# Autodesk Inventor assembly: ensambaje
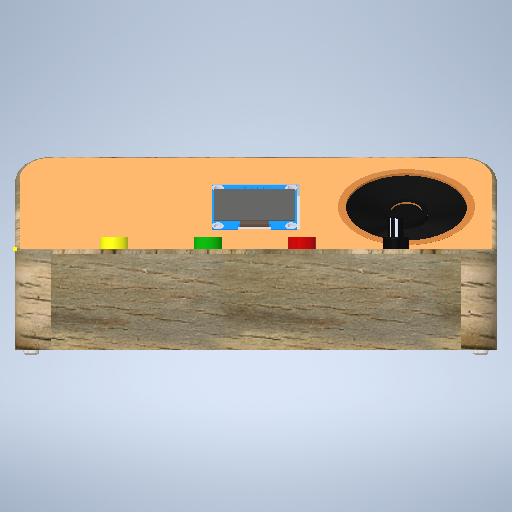
[picture p0: Inventor's stored thumbnail of the model, 512x512]
Saved by Autodesk Inventor 2025.3 (Build 293356000, 356)
## iProperties
Created: 2025-12-16
Part Number: ensambaje
Document SubType Name: Assembly
Designer: ar287
Author: ar287
## Documents named in this file (12)
- C:\Users\ar287\OneDrive - Escuela Superior Politécnica del Litoral\EMBEBIDOS\tarea4\ensambaje.iam
- C:\Users\ar287\OneDrive - Escuela Superior Politécnica del Litoral\EMBEBIDOS\tarea4\base.ipt
- C:\Users\ar287\Downloads\oled-1-3-128x64-1.snapshot.10\step\oled\oled\oledoled.ipt
- C:\Users\ar287\Downloads\bocina_57mm-1.snapshot.1\Bocina_57mm\Bocina_57mm\bocinaBocina_57mm.ipt
- C:\Users\ar287\OneDrive - Escuela Superior Politécnica del Litoral\EMBEBIDOS\tarea4\boton amarillo.ipt
- C:\Users\ar287\OneDrive - Escuela Superior Politécnica del Litoral\EMBEBIDOS\tarea4\boton rojo.ipt
- C:\Users\ar287\OneDrive - Escuela Superior Politécnica del Litoral\EMBEBIDOS\tarea4\boton verde.ipt
- C:\Users\ar287\OneDrive - Escuela Superior Politécnica del Litoral\EMBEBIDOS\tarea4\estuche de pot.ipt
- C:\Users\ar287\OneDrive - Escuela Superior Politécnica del Litoral\EMBEBIDOS\tarea4\pot.ipt
- C:\Users\ar287\Downloads\esp32-c6-wroom-1-1.snapshot.2\ESP32C6\ESP32C6\espESP32C6.iam
- C:\Users\ar287\Downloads\dfplayer-mini-3.snapshot.1\DFPlayer Mini Assem v1\DFPlayer Mini Assem v1\dfDFPlayer Mini Assem v1.iam
- C:\Users\ar287\OneDrive\Documentos\Inventor\Content Center Files\R2025\es-ES\DIN 7985 (Z)\DIN 7985 (Z) - M2,5x3-Z.ipt
## Components (21 placed, 11 different names)
1. base:1 — Coincidencia:1, Coincidencia:2, Coincidencia:3, Insertar:1, Coincidencia:4, Coincidencia:5, Nivelación:1, Insertar:2, Nivelación:2, Insertar:3, Nivelación:3, Insertar:4, Coincidencia:7, Insertar:6, Coincidencia:8, Coincidencia:9, Coincidencia:10, Coincidencia:11, Coincidencia:12, Coincidencia:13, Insertar:7, Insertar:8, Insertar:9, Insertar:10, Insertar:11, Coincidencia:14, Coincidencia:15, Coincidencia:16, Coincidencia:17, Coincidencia:18, Coincidencia:19, Coincidencia:20, Coincidencia:21, Coincidencia:22, Coincidencia:23, Coincidencia:24, Coincidencia:25
2. oledoled:1 — Coincidencia:1, Coincidencia:2, Coincidencia:3, Coincidencia:5
3. bocinaBocina_57mm:1 — Insertar:1, Coincidencia:4
4. boton amarillo:1 — Nivelación:1, Insertar:2
5. boton rojo:1 — Nivelación:3, Insertar:4
6. boton verde:1 — Nivelación:2, Insertar:3
7. estuche de pot:1 — Coincidencia:6, Insertar:5, Coincidencia:7, Insertar:6
8. pot:1 — Coincidencia:6, Insertar:5
9. espESP32C6:1 [sub-assembly] — Coincidencia:8, Coincidencia:9, Coincidencia:10
10. dfDFPlayer Mini Assem v1:1 [sub-assembly] — Coincidencia:11, Coincidencia:12, Coincidencia:13
11. DIN 7985 (Z) M2,5x3-Z:1 — Insertar:7
12. DIN 7985 (Z) M2,5x3-Z:2 — Insertar:8
13. DIN 7985 (Z) M2,5x3-Z:3 — Insertar:9
14. DIN 7985 (Z) M2,5x3-Z:4 — Insertar:10
15. DIN 7985 (Z) M2,5x3-Z:5 — Insertar:11
16. DIN 7985 (Z) M2,5x3-Z:6 — Coincidencia:14, Coincidencia:15
17. DIN 7985 (Z) M2,5x3-Z:7 — Coincidencia:16, Coincidencia:17
18. DIN 7985 (Z) M2,5x3-Z:8 — Coincidencia:18, Coincidencia:19
19. DIN 7985 (Z) M2,5x3-Z:9 — Coincidencia:20, Coincidencia:21
20. DIN 7985 (Z) M2,5x3-Z:10 — Coincidencia:22, Coincidencia:23
21. DIN 7985 (Z) M2,5x3-Z:11 — Coincidencia:24, Coincidencia:25
## Relationships (39: Mate 25, Insert 11, Flush 3)
- Coincidencia:1 [Mate]: base:1 ↔ oledoled:1
- Coincidencia:2 [Mate]: base:1 ↔ oledoled:1
- Coincidencia:3 [Mate]: base:1 ↔ oledoled:1
- Insertar:1 (-12 mm): base:1 ↔ bocinaBocina_57mm:1
- Coincidencia:4 [Mate]: base:1 ↔ bocinaBocina_57mm:1
- Coincidencia:5 [Mate]: base:1 ↔ oledoled:1
- Nivelación:1 [Flush]: base:1 ↔ boton amarillo:1
- Insertar:2: base:1 ↔ boton amarillo:1
- Nivelación:2 [Flush]: base:1 ↔ boton verde:1
- Insertar:3: base:1 ↔ boton verde:1
- Nivelación:3 [Flush]: base:1 ↔ boton rojo:1
- Insertar:4: base:1 ↔ boton rojo:1
- Coincidencia:6 [Mate]: estuche de pot:1 ↔ pot:1
- Insertar:5: estuche de pot:1 ↔ pot:1
- Coincidencia:7 [Mate]: base:1 ↔ estuche de pot:1
- Insertar:6: base:1 ↔ estuche de pot:1
- Coincidencia:8 [Mate]: base:1 ↔ espESP32C6:1
- Coincidencia:9 [Mate] (100 mm): base:1 ↔ espESP32C6:1
- Coincidencia:10 [Mate] (20 mm): base:1 ↔ espESP32C6:1
- Coincidencia:11 [Mate]: base:1 ↔ dfDFPlayer Mini Assem v1:1
- Coincidencia:12 [Mate] (50 mm): base:1 ↔ dfDFPlayer Mini Assem v1:1
- Coincidencia:13 [Mate] (20 mm): base:1 ↔ dfDFPlayer Mini Assem v1:1
- Insertar:7: base:1 ↔ DIN 7985 (Z) M2,5x3-Z:1
- Insertar:8: base:1 ↔ DIN 7985 (Z) M2,5x3-Z:2
- Insertar:9: base:1 ↔ DIN 7985 (Z) M2,5x3-Z:3
- Insertar:10: base:1 ↔ DIN 7985 (Z) M2,5x3-Z:4
- Insertar:11: base:1 ↔ DIN 7985 (Z) M2,5x3-Z:5
- Coincidencia:14 [Mate]: base:1 ↔ DIN 7985 (Z) M2,5x3-Z:6
- Coincidencia:15 [Mate]: base:1 ↔ DIN 7985 (Z) M2,5x3-Z:6
- Coincidencia:16 [Mate]: base:1 ↔ DIN 7985 (Z) M2,5x3-Z:7
- Coincidencia:17 [Mate]: base:1 ↔ DIN 7985 (Z) M2,5x3-Z:7
- Coincidencia:18 [Mate]: base:1 ↔ DIN 7985 (Z) M2,5x3-Z:8
- Coincidencia:19 [Mate]: base:1 ↔ DIN 7985 (Z) M2,5x3-Z:8
- Coincidencia:20 [Mate]: base:1 ↔ DIN 7985 (Z) M2,5x3-Z:9
- Coincidencia:21 [Mate]: base:1 ↔ DIN 7985 (Z) M2,5x3-Z:9
- Coincidencia:22 [Mate]: base:1 ↔ DIN 7985 (Z) M2,5x3-Z:10
- Coincidencia:23 [Mate]: base:1 ↔ DIN 7985 (Z) M2,5x3-Z:10
- Coincidencia:24 [Mate]: base:1 ↔ DIN 7985 (Z) M2,5x3-Z:11
- Coincidencia:25 [Mate]: base:1 ↔ DIN 7985 (Z) M2,5x3-Z:11
